# Autodesk Inventor assembly: Assembly4
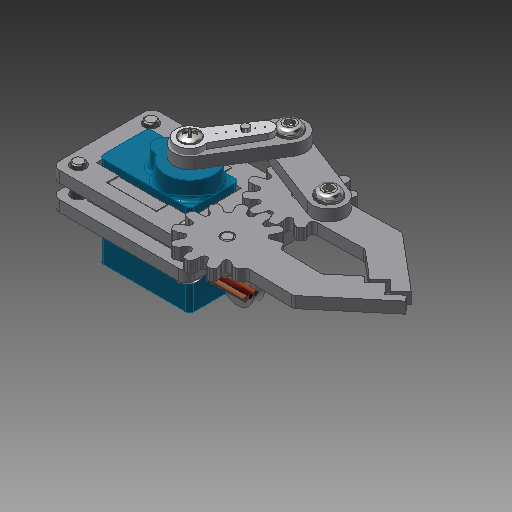
[picture p0: Inventor's stored thumbnail of the model, 512x512]
Saved by Autodesk Inventor 2019.2 (Build 232265000, 265)
## iProperties
Created: 2019-04-05
Part Number: Assembly4
Document SubType Name: Assembly
Designer: richard.girt
Mass: 21.3293 g
Surface Area: 131.622 cm^2
Volume: 15.4863 cm^3
Density: 1.3773 g/cm^3
Author: richard.girt
## Documents named in this file (16)
- C:\Users\richard.girt\Desktop\2 Axis robotic arm\Assembly4.iam
- C:\Users\richard.girt\Desktop\2 Axis robotic arm\SG90.ipt
- C:\Users\richard.girt\Desktop\2 Axis robotic arm\Part17.ipt
- C:\Users\richard.girt\Desktop\2 Axis robotic arm\Part19.ipt
- C:\Users\richard.girt\Desktop\2 Axis robotic arm\Part18.ipt
- C:\Users\richard.girt\Desktop\2 Axis robotic arm\Part20.ipt
- C:\Users\richard.girt\Desktop\2 Axis robotic arm\Part21.ipt
- C:\Users\richard.girt\Desktop\2 Axis robotic arm\Part22.ipt
- C:\Users\richard.girt\Desktop\2 Axis robotic arm\SG90Horn1.ipt
- C:\Users\richard.girt\Desktop\2 Axis robotic arm\ANSI B18.6.5M - M2.5x0.45 x 4(38).ipt
- C:\Users\richard.girt\Desktop\2 Axis robotic arm\ANSI B18.6.5M - M2.5x0.45 x 8(38).ipt
- ANSI B18.6.5M - M2.5x0.45 x 8(38).ipt
- C:\Users\richard.girt\Desktop\2 Axis robotic arm\Part23.ipt
- C:\Users\richard.girt\Desktop\2 Axis robotic arm\Part25.ipt
- C:\Users\richard.girt\Desktop\2 Axis robotic arm\ANSI B18.3.4M - M3 x 0.5 x 8(1).ipt
- C:\_Vault\Content Center\en-US\ANSI B18.3.4M(2)\ANSI B18.3.4M - M3 x 0.5 x 6(1).ipt
## Components (20 placed, 14 different names)
1. SG90:1 — Mate:2, Mate:3, Flush:6, Flush:7, Mate:9, Mate:10, Mate:14, Rotational:1
2. Part17:1 — Mate:2, Mate:3, Mate:4, Mate:5, Mate:6, Mate:7, Mate:12, Mate:13, Mate:14, Mate:17, Rigid:6, Rigid:7
3. Part19:1 — Mate:6, Mate:7, Flush:7, Mate:8
4. Part18:1 — Mate:4, Flush:6, Mate:5
5. Part20:1 — Mate:8, Mate:9, Mate:10, Rigid:4, Rotational:2, Rotational:3, Rigid:5
6. Part21:1 — Flush:8, Mate:11, Mate:13, Symmetry:1, Mate:17
7. Part22:1 — Flush:8, Mate:11, Mate:12, Symmetry:1, Mate:16, Mate:18
8. Part23:1 — Rigid:1, Mate:15, Rigid:9
9. SG90Horn1:1 — Rigid:1, Rotational:1
10. ANSI B18.6.5M - M2.5x0.45 x 4(38):1
11. ANSI B18.6.5M - M2.5x0.45 x 8(38):1
12. Part25:1 — Mate:15, Mate:16, Mate:18, Rigid:8
13. ANSI B18.3.4M - M3 x 0.5 x 8(1):1 — Rigid:5
14. ANSI B18.3.4M - M3 x 0.5 x 8(1):3 — Rigid:4
15. ANSI B18.3.4M - M3 x 0.5 x 8(1):4 — Rotational:2
16. ANSI B18.3.4M - M3 x 0.5 x 8(1):2 — Rotational:3
17. Forged Hexagon Socket Button Head Cap Screw - Metric M3 x 0.5 x 6:2 — Rigid:6
18. Forged Hexagon Socket Button Head Cap Screw - Metric M3 x 0.5 x 6:3 — Rigid:7
19. Forged Hexagon Socket Button Head Cap Screw - Metric M3 x 0.5 x 6:4 — Rigid:8
20. Forged Hexagon Socket Button Head Cap Screw - Metric M3 x 0.5 x 6:5 — Rigid:9
## Relationships (33: Mate 17, WeldJoint 9, Flush 3, RevoluteJoint 3, Symmetry 1)
- Mate:2: SG90:1 ↔ Part17:1
- Mate:3: SG90:1 ↔ Part17:1
- Mate:4: Part17:1 ↔ Part18:1
- Flush:6: SG90:1 ↔ Part18:1
- Mate:5: Part17:1 ↔ Part18:1
- Mate:6: Part17:1 ↔ Part19:1
- Mate:7: Part17:1 ↔ Part19:1
- Flush:7: SG90:1 ↔ Part19:1
- Mate:8: Part19:1 ↔ Part20:1
- Mate:9: SG90:1 ↔ Part20:1
- Mate:10: SG90:1 ↔ Part20:1
- Flush:8: Part21:1 ↔ Part22:1
- Mate:11 (18 mm): Part21:1 ↔ Part22:1
- Mate:12: Part17:1 ↔ Part22:1
- Mate:13: Part17:1 ↔ Part21:1
- Symmetry:1: Part21:1 ↔ Part22:1
- Mate:14: SG90:1 ↔ Part17:1
- Rigid:1 [WeldJoint]: Part23:1 ↔ SG90Horn1:1
- [WeldJoint]: SG90Horn1:1 ↔ ANSI B18.6.5M - M2.5x0.45 x 4(38):1
- [WeldJoint] (-2.8 mm): SG90Horn1:1 ↔ ANSI B18.6.5M - M2.5x0.45 x 8(38):1
- Rotational:1 [RevoluteJoint]: SG90:1 ↔ SG90Horn1:1
- Mate:15: Part23:1 ↔ Part25:1
- Mate:16: Part22:1 ↔ Part25:1
- Mate:17 (0.3367 mm): Part17:1 ↔ Part21:1
- Mate:18 (0.3367 mm): Part22:1 ↔ Part25:1
- Rigid:4 [WeldJoint]: Part20:1 ↔ ANSI B18.3.4M - M3 x 0.5 x 8(1):3
- Rotational:2 [RevoluteJoint]: Part20:1 ↔ ANSI B18.3.4M - M3 x 0.5 x 8(1):4
- Rotational:3 [RevoluteJoint]: Part20:1 ↔ ANSI B18.3.4M - M3 x 0.5 x 8(1):2
- Rigid:5 [WeldJoint]: Part20:1 ↔ ANSI B18.3.4M - M3 x 0.5 x 8(1):1
- Rigid:6 [WeldJoint]: Part17:1 ↔ Forged Hexagon Socket Button Head Cap Screw - Metric M3 x 0.5 x 6:2
- Rigid:7 [WeldJoint]: Part17:1 ↔ Forged Hexagon Socket Button Head Cap Screw - Metric M3 x 0.5 x 6:3
- Rigid:8 [WeldJoint]: Part25:1 ↔ Forged Hexagon Socket Button Head Cap Screw - Metric M3 x 0.5 x 6:4
- Rigid:9 [WeldJoint]: Part23:1 ↔ Forged Hexagon Socket Button Head Cap Screw - Metric M3 x 0.5 x 6:5
